# Autodesk Inventor assembly: fly_funnel_combinations
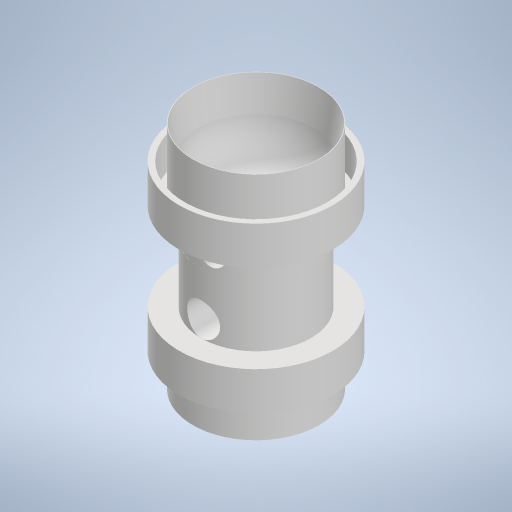
[picture p0: Inventor's stored thumbnail of the model, 512x512]
Saved by Autodesk Inventor 2023.1 (Build 271208000, 208)
## iProperties
Created: 2023-05-01
Part Number: fly_funnel_combinations
Document SubType Name: Assembly
Designer: dinesh
Author: dinesh
## Documents named in this file (3)
- C:\Users\dinesh\Dropbox\Desktop_Sync\Inventor_Projects\custom_designs\fly_funnel\fly_funnel_combinations.iam
- C:\Users\dinesh\Dropbox\Desktop_Sync\Inventor_Projects\custom_designs\fly_funnel\vial_adapter_female.ipt
- C:\Users\dinesh\Dropbox\Desktop_Sync\Inventor_Projects\custom_designs\fly_funnel\vial_adapter_male.ipt
## Components (2 placed, 2 different names)
1. vial_adapter_female:1 — Mate:1, Mate:2
2. vial_adapter_male:1 — Mate:1, Mate:2
## Relationships (2: Mate 2)
- Mate:1: vial_adapter_female:1 ↔ vial_adapter_male:1
- Mate:2: vial_adapter_female:1 ↔ vial_adapter_male:1
